# Autodesk Inventor assembly: TPU Based Assembly
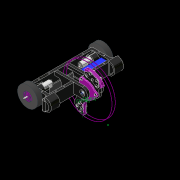
[picture p0: Inventor's stored thumbnail of the model, 180x180]
Saved by Autodesk Inventor 2022 (Build 260153000, 153)
## iProperties
Created: 2022-02-23
Part Number: TPU Based Assembly
Document SubType Name: Assembly
Designer: tandu
Mass: 377.258 g
Surface Area: 1147.57 cm^2
Volume: 253.768 cm^3
Density: 1.48663 g/cm^3
Author: tandu
## Documents named in this file (10)
- C:\Users\tandu\Documents\GrabCAD\Insomnia 2020\Versions\7 New form 6 20 22\TPU Based Assembly 7.iam
- C:\Users\tandu\Documents\GrabCAD\Insomnia 2020\Versions\7 New form 6 20 22\BatteryMockup.ipt
- C:\Users\tandu\Documents\GrabCAD\Insomnia 2020\Versions\7 New form 6 20 22\CorrectSizeWheelsIThink.ipt
- C:\Users\tandu\Documents\GrabCAD\Insomnia 2020\Versions\7 New form 6 20 22\EMax RS2205 v1.ipt
- C:\Users\tandu\Documents\GrabCAD\Insomnia 2020\Versions\7 New form 6 20 22\FingerTech_Silver_Spark_223350.ipt
- C:\Users\tandu\Documents\GrabCAD\Insomnia 2020\Versions\7 New form 6 20 22\TPU 22 Chassis.ipt
- C:\Users\tandu\Documents\GrabCAD\Insomnia 2020\Versions\7 New form 6 20 22\UHMWMotorUpright.ipt
- C:\Users\tandu\Documents\GrabCAD\Insomnia 2020\Versions\7 New form 6 20 22\UHMWBearingUpright.ipt
- C:\Users\tandu\Documents\GrabCAD\Insomnia 2020\Versions\7 New form 6 20 22\57155K571_Flanged Ball Bearing.ipt
- C:\Users\tandu\Documents\GrabCAD\Insomnia 2020\Versions\6 Better liveshaft weapon 5 13 22\Weapon\Aluminimumanfmonfo Jank Weapon Fix.iam
## Components (11 placed, 9 different names)
1. BatteryMockup:1 — Mate:1, Mate:2, Mate:3
2. CorrectSizeWheelsIThink:1 — Insert:2
3. FingerTech_Silver_Spark_223350:1 — Insert:9, Mate:4
4. TPU 22 Chassis:1 — Mate:1, Mate:2, Mate:3, Insert:1, Insert:2, Insert:9, Mate:4, Insert:10, Mate:5, Insert:11, Insert:12, Insert:13, Insert:14
5. FingerTech_Silver_Spark_223350:2 — Insert:10, Mate:5
6. CorrectSizeWheelsIThink:2 — Insert:1
7. UHMWMotorUpright:1 — Insert:11, Insert:12, Insert:15, Insert:16
8. UHMWBearingUpright:1 — Insert:13, Insert:14, Insert:22
9. EMax RS2205 v1:1 — Insert:15, Insert:16, Insert:23
10. 57155K571_Flanged Ball Bearing:1 — Insert:22
11. Aluminimumanfmonfo Jank Weapon Fix:1 [sub-assembly] — Insert:23
## Relationships (17: Insert 12, Mate 5)
- Mate:1: BatteryMockup:1 ↔ TPU 22 Chassis:1
- Mate:2: BatteryMockup:1 ↔ TPU 22 Chassis:1
- Mate:3: BatteryMockup:1 ↔ TPU 22 Chassis:1
- Insert:1: TPU 22 Chassis:1 ↔ CorrectSizeWheelsIThink:2
- Insert:2: CorrectSizeWheelsIThink:1 ↔ TPU 22 Chassis:1
- Insert:9: FingerTech_Silver_Spark_223350:1 ↔ TPU 22 Chassis:1
- Mate:4: FingerTech_Silver_Spark_223350:1 ↔ TPU 22 Chassis:1
- Insert:10: TPU 22 Chassis:1 ↔ FingerTech_Silver_Spark_223350:2
- Mate:5: TPU 22 Chassis:1 ↔ FingerTech_Silver_Spark_223350:2
- Insert:11: TPU 22 Chassis:1 ↔ UHMWMotorUpright:1
- Insert:12: TPU 22 Chassis:1 ↔ UHMWMotorUpright:1
- Insert:13: TPU 22 Chassis:1 ↔ UHMWBearingUpright:1
- Insert:14: TPU 22 Chassis:1 ↔ UHMWBearingUpright:1
- Insert:15: UHMWMotorUpright:1 ↔ EMax RS2205 v1:1
- Insert:16: UHMWMotorUpright:1 ↔ EMax RS2205 v1:1
- Insert:22: UHMWBearingUpright:1 ↔ 57155K571_Flanged Ball Bearing:1
- Insert:23: EMax RS2205 v1:1 ↔ Aluminimumanfmonfo Jank Weapon Fix:1
